# Autodesk Inventor assembly: truefit
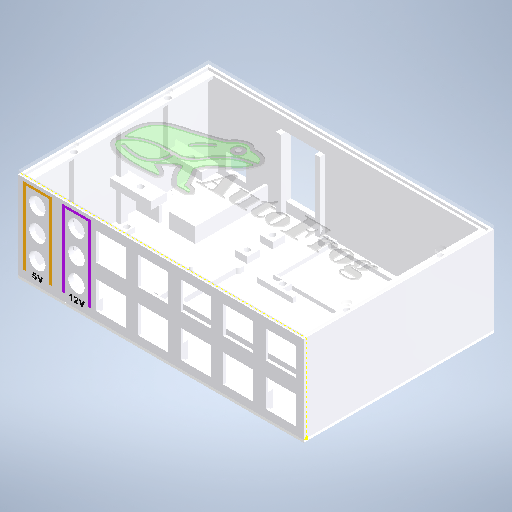
[picture p0: Inventor's stored thumbnail of the model, 512x512]
Saved by Autodesk Inventor 2025 (Build 290162000, 162)
## iProperties
Created: 2025-05-15
Part Number: truefit
Document SubType Name: Assembly
Designer: ethan
Author: ethan
## Documents named in this file (7)
- C:\Users\ethan\Documents\GitHub\AutoFrog2\CAD\truefit.iam
- C:\Users\ethan\Documents\GitHub\AutoFrog2\CAD\case\baseplate.ipt
- C:\Users\ethan\Documents\GitHub\AutoFrog2\CAD\case\leftwall.ipt
- C:\Users\ethan\Documents\GitHub\AutoFrog2\CAD\case\rightwall.ipt
- C:\Users\ethan\Documents\GitHub\AutoFrog2\CAD\case\frontpanel.ipt
- C:\Users\ethan\Documents\GitHub\AutoFrog2\CAD\case\backplate.ipt
- C:\Users\ethan\Documents\GitHub\AutoFrog2\CAD\case\Lid.ipt
## Components (6 placed, 6 different names)
1. baseplate:1 — Mate:1, Mate:4, Mate:8, Mate:9, Mate:10, Flush:1, Flush:2, Flush:3, Mate:13, Mate:14
2. leftwall:1 — Mate:1, Mate:9, Flush:3, Mate:12, Mate:15
3. rightwall:1 — Mate:4, Mate:10, Flush:2, Flush:5, Flush:6
4. frontpanel:1 — Mate:8, Flush:1, Mate:13
5. backplate:1 — Mate:12, Mate:14, Mate:15
6. Lid:1 — Flush:5, Flush:6
## Relationships (14: Mate 9, Flush 5)
- Mate:1: baseplate:1 ↔ leftwall:1
- Mate:4: baseplate:1 ↔ rightwall:1
- Mate:8: baseplate:1 ↔ frontpanel:1
- Mate:9: baseplate:1 ↔ leftwall:1
- Mate:10: baseplate:1 ↔ rightwall:1
- Flush:1: baseplate:1 ↔ frontpanel:1
- Flush:2: baseplate:1 ↔ rightwall:1
- Flush:3: baseplate:1 ↔ leftwall:1
- Mate:12: leftwall:1 ↔ backplate:1
- Mate:13: baseplate:1 ↔ frontpanel:1
- Mate:14: baseplate:1 ↔ backplate:1
- Flush:5: rightwall:1 ↔ Lid:1
- Flush:6: rightwall:1 ↔ Lid:1
- Mate:15: leftwall:1 ↔ backplate:1
